# Autodesk Inventor assembly: Assembly1
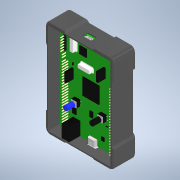
[picture p0: Inventor's stored thumbnail of the model, 180x180]
Saved by Autodesk Inventor 2020 (Build 240168000, 168)
## iProperties
Created: 2025-03-09
Part Number: Assembly1
Document SubType Name: Assembly
Designer: mahun
Author: mahun
## Documents named in this file (3)
- C:\Users\mahun\Desktop\MINBOT LABS\PROJECT\Hoc STM32F411VET6\Case for STM32F4-Discovery Board\Assembly1.iam
- C:\Users\mahun\Desktop\MINBOT LABS\PROJECT\Hoc STM32F411VET6\Case for STM32F4-Discovery Board\case.ipt
- C:\Users\mahun\Desktop\MINBOT LABS\PROJECT\Hoc STM32F411VET6\Case for STM32F4-Discovery Board\stm32f411EDISCO.ipt
## Components (2 placed, 2 different names)
1. case:1 — Mate:1, Mate:2, Mate:3
2. stm32f411EDISCO:1 — Mate:1, Mate:2, Mate:3
## Relationships (3: Mate 3)
- Mate:1: case:1 ↔ stm32f411EDISCO:1
- Mate:2: case:1 ↔ stm32f411EDISCO:1
- Mate:3: case:1 ↔ stm32f411EDISCO:1
